# Autodesk Inventor assembly: Assembly1
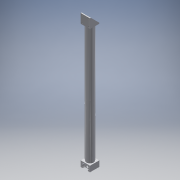
[picture p0: Inventor's stored thumbnail of the model, 180x180]
Saved by Autodesk Inventor 2016 (Build 200138000, 138)
## iProperties
Created: 2017-05-27
Part Number: Assembly1
Document SubType Name: Assembly
Designer: Kyle
Mass: 216.598 g
Surface Area: 799.465 cm^2
Volume: 80.2217 cm^3
Density: 2.7 g/cm^3
Author: Kyle
## Documents named in this file (4)
- C:\Users\Kyle\Documents\inverted pendulum\Assembly1.iam
- C:\Users\Kyle\Documents\inverted pendulum\bearingholder.ipt
- C:\Users\Kyle\Documents\inverted pendulum\tube.ipt
- C:\Users\Kyle\Documents\inverted pendulum\motormount.ipt
## Components (3 placed, 3 different names)
1. bearingholder:1 — Mate:1, Mate:2, Angle:1
2. tube:1 — Mate:1, Mate:2, Mate:3, Mate:4
3. motormount:1 — Mate:3, Mate:4, Angle:1
## Relationships (5: Mate 4, Angle 1)
- Mate:1: bearingholder:1 ↔ tube:1
- Mate:2: bearingholder:1 ↔ tube:1
- Mate:3: tube:1 ↔ motormount:1
- Mate:4: tube:1 ↔ motormount:1
- Angle:1 (0 deg): bearingholder:1 ↔ motormount:1
